# Autodesk Inventor assembly: STARduino and Pi assembly
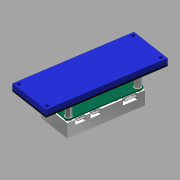
[picture p0: Inventor's stored thumbnail of the model, 180x180]
Saved by Autodesk Inventor 2017 (Build 210142000, 142)
## iProperties
Created: 2017-01-16
Part Number: STARduino and Pi assembly
Document SubType Name: Assembly
Designer: qupec
Author: qupec
## Documents named in this file (6)
- C:\Users\qupec\Desktop\UMD Near Space\STAR\CAD\Mechanical\STARduino and Pi assembly.iam
- C:\Users\qupec\Desktop\UMD Near Space\STAR\CAD\Mechanical\STARduino layout.ipt
- C:\Users\qupec\Desktop\UMD Near Space\STAR\CAD\Mechanical\STARduino Mount.ipt
- C:\Users\qupec\Desktop\UMD Near Space\STAR\CAD\Mechanical\Pi Cam\RapberryPiZero.ipt
- C:\Users\qupec\Desktop\UMD Near Space\STAR\CAD\Mechanical\Standoff for Pi.ipt
- C:\Users\qupec\Desktop\UMD Near Space\STAR\CAD\Mechanical\Heat Block for Pi.ipt
## Components (8 placed, 5 different names)
1. STARduino layout:1 — Mate:7, Mate:12, Mate:13, Mate:14, Mate:15, Mate:16, Mate:17, Mate:18, Mate:19, Mate:23, Mate:24
2. STARduino Mount:1 — Mate:7, Mate:23, Mate:24
3. RapberryPiZero:1 — Mate:20, Mate:21, Mate:22, Mate:25, Mate:26, Mate:27
4. Standoff for Pi:1 — Mate:13, Mate:17, Mate:22
5. Standoff for Pi:2 — Mate:12, Mate:18
6. Standoff for Pi:3 — Mate:15, Mate:16
7. Standoff for Pi:4 — Mate:14, Mate:19, Mate:20, Mate:21
8. Heat Block for Pi:1 — Mate:25, Mate:26, Mate:27
## Relationships (17: Mate 17)
- Mate:7: STARduino layout:1 ↔ STARduino Mount:1
- Mate:12: STARduino layout:1 ↔ Standoff for Pi:2
- Mate:13: STARduino layout:1 ↔ Standoff for Pi:1
- Mate:14: STARduino layout:1 ↔ Standoff for Pi:4
- Mate:15: STARduino layout:1 ↔ Standoff for Pi:3
- Mate:16: STARduino layout:1 ↔ Standoff for Pi:3
- Mate:17: STARduino layout:1 ↔ Standoff for Pi:1
- Mate:18: STARduino layout:1 ↔ Standoff for Pi:2
- Mate:19: STARduino layout:1 ↔ Standoff for Pi:4
- Mate:20: RapberryPiZero:1 ↔ Standoff for Pi:4
- Mate:21: RapberryPiZero:1 ↔ Standoff for Pi:4
- Mate:22: RapberryPiZero:1 ↔ Standoff for Pi:1
- Mate:23: STARduino layout:1 ↔ STARduino Mount:1
- Mate:24: STARduino layout:1 ↔ STARduino Mount:1
- Mate:25: RapberryPiZero:1 ↔ Heat Block for Pi:1
- Mate:26: RapberryPiZero:1 ↔ Heat Block for Pi:1
- Mate:27: RapberryPiZero:1 ↔ Heat Block for Pi:1
